# Autodesk Inventor assembly: Elektro_asm
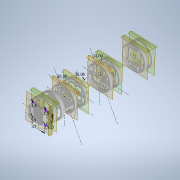
[picture p0: Inventor's stored thumbnail of the model, 180x180]
Saved by Autodesk Inventor 2020 (Build 240168000, 168)
## iProperties
Created: 2022-03-10
Part Number: Elektro_asm
Document SubType Name: Assembly
Designer: sp
Author: sp
## Documents named in this file (10)
- C:\Users\sp\Documents\Rocket\rocket\CAD\Elektro_asm.iam
- C:\Users\sp\Documents\Rocket\rocket\CAD\Electro_unit.ipt
- C:\Users\sp\Documents\Rocket\rocket\CAD\Elektro_Gyro.ipt
- C:\Users\sp\Documents\Rocket\rocket\CAD\Electro_gps.ipt
- C:\Users\sp\Documents\Rocket\rocket\CAD\Electro_bat_down.ipt
- C:\Users\sp\Documents\Rocket\rocket\CAD\Electro_bat_up.ipt
- C:\Users\sp\Documents\Rocket\rocket\CAD\Electro_esp32.ipt
- C:\Users\sp\Documents\Rocket\rocket\CAD\Electro_esp32_up.ipt
- C:\Users\sp\Documents\Rocket\rocket\CAD\Electro_Sensor.ipt
- C:\Users\sp\Documents\Rocket\rocket\CAD\Electro_lora.ipt
## Components (9 placed, 9 different names)
1. Electro_unit:1 — Einfügen:5, Passend:4
2. Elektro_Gyro:1 — Einfügen:3, Einfügen:11, Passend:9, Passend:10, Fluchtend:1
3. Electro_gps:1 — Einfügen:3, Passend:9, Passend:11
4. Electro_bat_down:1 — Einfügen:6, Einfügen:8, Passend:5, Passend:6
5. Electro_bat_up:1 — Einfügen:5, Einfügen:8, Passend:4, Passend:5
6. Electro_esp32:1 — Einfügen:6, Einfügen:9, Passend:6, Passend:7
7. Electro_esp32_up:1 — Einfügen:9, Einfügen:10, Passend:7, Passend:8
8. Electro_Sensor:1 — Einfügen:10, Einfügen:11, Passend:8, Passend:10
9. Electro_lora:1 — Passend:11, Fluchtend:1
## Relationships (16: Mate 8, Insert 7, Flush 1)
- Einfügen:3 [Insert] (10 mm): Elektro_Gyro:1 ↔ Electro_gps:1
- Einfügen:5 [Insert] (10 mm): Electro_unit:1 ↔ Electro_bat_up:1
- Einfügen:6 [Insert] (15 mm): Electro_bat_down:1 ↔ Electro_esp32:1
- Einfügen:8 [Insert] (59 mm): Electro_bat_down:1 ↔ Electro_bat_up:1
- Einfügen:9 [Insert] (56 mm): Electro_esp32:1 ↔ Electro_esp32_up:1
- Einfügen:10 [Insert] (20 mm): Electro_esp32_up:1 ↔ Electro_Sensor:1
- Einfügen:11 [Insert] (26 mm): Elektro_Gyro:1 ↔ Electro_Sensor:1
- Passend:4 [Mate]: Electro_unit:1 ↔ Electro_bat_up:1
- Passend:5 [Mate]: Electro_bat_down:1 ↔ Electro_bat_up:1
- Passend:6 [Mate]: Electro_bat_down:1 ↔ Electro_esp32:1
- Passend:7 [Mate]: Electro_esp32:1 ↔ Electro_esp32_up:1
- Passend:8 [Mate]: Electro_esp32_up:1 ↔ Electro_Sensor:1
- Passend:9 [Mate]: Elektro_Gyro:1 ↔ Electro_gps:1
- Passend:10 [Mate]: Elektro_Gyro:1 ↔ Electro_Sensor:1
- Passend:11 [Mate] (10 mm): Electro_gps:1 ↔ Electro_lora:1
- Fluchtend:1 [Flush]: Elektro_Gyro:1 ↔ Electro_lora:1
